# Autodesk Inventor assembly: Valve2.5
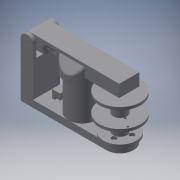
[picture p0: Inventor's stored thumbnail of the model, 180x180]
Saved by Autodesk Inventor 2019 (Build 230136000, 136)
## iProperties
Created: 2019-02-21
Part Number: Valve2.5
Document SubType Name: Assembly
Designer: Kepler
Author: Kepler
## Documents named in this file (5)
- C:\Users\Kepler\Documents\Inventor\Organ Valves\OrganValveMk2\Valve2.5.iam
- C:\Users\Kepler\Documents\Inventor\Organ Valves\OrganValveMk2\ValveBaseMk2.4.ipt
- C:\Users\Kepler\Documents\Inventor\Organ Valves\OrganValveMk2\Axel Mk2.ipt
- C:\Users\Kepler\Documents\Inventor\Organ Valves\OrganValveMk2\ValveHeadMk2.4.ipt
- C:\Users\Kepler\Documents\Inventor\Organ Valves\OrganValveMk2\SpoolMk2.ipt
## Components (4 placed, 4 different names)
1. ValveBaseMk2.4:1 — Insert:1, Mate:1, Mate:2, Mate:3, Mate:4
2. Axel Mk2:1 — Insert:1
3. ValveHeadMk2.4:1 — Mate:1, Mate:2
4. SpoolMk2:1 — Mate:3, Mate:4
## Relationships (5: Mate 4, Insert 1)
- Insert:1: ValveBaseMk2.4:1 ↔ Axel Mk2:1
- Mate:1 (0.1 mm): ValveBaseMk2.4:1 ↔ ValveHeadMk2.4:1
- Mate:2: ValveBaseMk2.4:1 ↔ ValveHeadMk2.4:1
- Mate:3: ValveBaseMk2.4:1 ↔ SpoolMk2:1
- Mate:4: ValveBaseMk2.4:1 ↔ SpoolMk2:1
